# Autodesk Inventor assembly: Construction
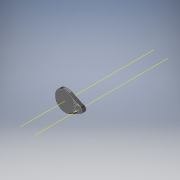
[picture p0: Inventor's stored thumbnail of the model, 180x180]
Saved by Autodesk Inventor 2018.3 (Build 223284000, 284)
## iProperties
Created: 2018-07-27
Part Number: Construction
Material: Generisch
Document SubType Name: Assembly
Designer: JochenAlt
Author: JochenAlt
## Documents named in this file (2)
- D:\Projects\Ondine\CAD\Beltdrive\Construction.iam
- D:\Projects\Ondine\CAD\Beltdrive\Construction\Übertragung des Zahnriemens4.iam
## Components (1 placed, 1 different names)
1. Übertragung des Zahnriemens:6 [sub-assembly] — Passend:2, Passend:3
## Relationships (2: Mate 2)
- Passend:2 [Mate]: Übertragung des Zahnriemens:6
- Passend:3 [Mate]: Übertragung des Zahnriemens:6
